# Autodesk Inventor assembly: frame
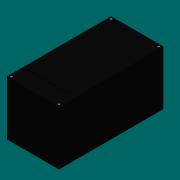
[picture p0: Inventor's stored thumbnail of the model, 180x180]
Saved by Autodesk Inventor 2016 SP1 (Build 200210100, 210)
## iProperties
Created: 2015-10-13
Part Number: frame
Document SubType Name: Assembly
Designer: Sawaiz
Author: Sawaiz
## Documents named in this file (16)
- C:\Users\sawai\OneDrive\projects\modularRICH\frame\frame.iam
- C:\Users\sawai\OneDrive\projects\modularRICH\frame\leftSide.ipt
- C:\Users\sawai\OneDrive\projects\modularRICH\frame\rightSide.ipt
- C:\Users\sawai\OneDrive\projects\modularRICH\frame\back.ipt
- C:\Users\sawai\OneDrive\projects\modularRICH\frame\bottom.ipt
- C:\Users\sawai\OneDrive\projects\modularRICH\frame\front.ipt
- C:\Users\sawai\OneDrive\projects\modularRICH\frame\top.ipt
- C:\Users\sawai\OneDrive\projects\modularRICH\hardware\4-40x0.5in.ipt
- C:\Users\sawai\OneDrive\projects\modularRICH\frame\topORing.ipt
- C:\Users\sawai\OneDrive\projects\modularRICH\dependency\modularRICHBackplane\cad\backplane.iam
- C:\Users\sawai\OneDrive\projects\modularRICH\hardware\no4nut.ipt
- C:\Users\sawai\OneDrive\projects\modularRICH\hardware\no4washer.ipt
- C:\Users\sawai\OneDrive\projects\modularRICH\connector\shv.ipt
- C:\Users\sawai\OneDrive\projects\modularRICH\connector\lvConnector.ipt
- C:\Users\sawai\OneDrive\projects\modularRICH\hardware\4-40x0.325in.ipt
- C:\Users\sawai\OneDrive\projects\modularRICH\modularRICH.xlsx
## Components (46 placed, 14 different names)
1. leftSide:1 — Flush:1, Flush:2, Flush:9, Flush:10
2. rightSide:1 — Flush:1, Flush:2, Flush:3, Flush:4, Flush:5, Mate:2, Flush:8, Mate:3
3. back:1 — Flush:4, Flush:8, Mate:3, Flush:11, Mate:36, Flush:22, Mate:37, Mate:38, Mate:39, Mate:40, Mate:41, Mate:42, Mate:43, Mate:69, Mate:72, Mate:73, Mate:74, Mate:75, Mate:76, Mate:77, Mate:78, Mate:79, Mate:80, Mate:81, Mate:82
4. bottom:1 — Flush:6, Mate:1, Flush:7
5. front:1 — Flush:3, Flush:5, Flush:6, Mate:1, Flush:7, Mate:2, Flush:9, Mate:11
6. top:1 — Flush:10, Flush:11, Mate:4, Mate:5, Mate:6, Mate:7, Flush:12, Flush:13, Flush:14, Flush:15, Mate:8, Mate:9, Mate:10, Mate:11
7. 4-40x0.5in:1 — Mate:4, Flush:15
8. 4-40x0.5in:2 — Mate:7, Flush:12
9. 4-40x0.5in:3 — Mate:6, Flush:13
10. 4-40x0.5in:4 — Mate:5, Flush:14
11. topORing:1 — Mate:8, Mate:9, Mate:10
12. 4-40x0.5in:5 — Mate:36, Flush:22, Flush:28, Flush:29, Mate:46
13. 4-40x0.5in:6 — Mate:37, Flush:29, Mate:66
14. 4-40x0.5in:7 — Mate:38, Flush:23, Mate:67
15. 4-40x0.5in:8 — Mate:42, Flush:27, Flush:28, Mate:62
16. 4-40x0.5in:9 — Mate:39, Flush:25, Flush:26, Mate:64
17. 4-40x0.5in:10 — Mate:40, Flush:26, Flush:27, Mate:63
18. 4-40x0.5in:11 — Mate:41, Flush:24, Flush:25, Mate:65
19. 4-40x0.5in:12 — Mate:43, Flush:23, Flush:24, Mate:68
20. no4nut:1 — Mate:44, Mate:45, Mate:46, Flush:30
21. no4washer:1 — Mate:44, Mate:45
22. no4nut:2 — Mate:64, Flush:35, Flush:36
23. no4washer:2 — Mate:71
24. no4nut:3 — Mate:63, Flush:36, Flush:37
25. no4washer:3
26. no4nut:4 — Mate:65, Flush:34, Flush:35
27. no4washer:4
28. no4nut:5 — Mate:67, Flush:32, Flush:33
29. no4washer:5
30. no4nut:6 — Mate:68, Flush:33, Flush:34
31. no4washer:6
32. no4nut:7 — Mate:66, Flush:31, Flush:32
33. no4washer:7
34. no4nut:8 — Mate:62, Flush:30, Flush:31, Flush:37
35. no4washer:8 — Mate:70
36. backplane:1 [sub-assembly] — Mate:69, Mate:70, Mate:71
37. shv:1 — Mate:72, Mate:73, Flush:38
38. shv:2 — Mate:74, Flush:38, Flush:40
39. shv:3 — Mate:75, Flush:39, Flush:40
40. shv:4 — Mate:76, Flush:39
41. lvConnector:1 — Mate:77, Mate:78, Mate:79, Mate:86, Mate:87, Mate:88, Mate:89
42. lvConnector:2 — Mate:80, Mate:81, Mate:82, Mate:83, Mate:84, Mate:85, Mate:90
43. 4-40x0.325in:1 — Mate:83, Mate:84
44. 4-40x0.325in:2 — Mate:85, Mate:90
45. 4-40x0.325in:3 — Mate:86, Mate:88
46. 4-40x0.325in:4 — Mate:87, Mate:89
## Relationships (99: Mate 65, Flush 34)
- Flush:1: leftSide:1 ↔ rightSide:1
- Flush:2: leftSide:1 ↔ rightSide:1
- Flush:3: rightSide:1 ↔ front:1
- Flush:4: rightSide:1 ↔ back:1
- Flush:5: rightSide:1 ↔ front:1
- Flush:6: bottom:1 ↔ front:1
- Mate:1: bottom:1 ↔ front:1
- Flush:7: bottom:1 ↔ front:1
- Mate:2: rightSide:1 ↔ front:1
- Flush:8: rightSide:1 ↔ back:1
- Mate:3: rightSide:1 ↔ back:1
- Flush:9: leftSide:1 ↔ front:1
- Flush:10: leftSide:1 ↔ top:1
- Flush:11: back:1 ↔ top:1
- Mate:4: top:1 ↔ 4-40x0.5in:1
- Mate:5: top:1 ↔ 4-40x0.5in:4
- Mate:6: top:1 ↔ 4-40x0.5in:3
- Mate:7: top:1 ↔ 4-40x0.5in:2
- Flush:12: top:1 ↔ 4-40x0.5in:2
- Flush:13: top:1 ↔ 4-40x0.5in:3
- Flush:14: top:1 ↔ 4-40x0.5in:4
- Flush:15: top:1 ↔ 4-40x0.5in:1
- Mate:8: top:1 ↔ topORing:1
- Mate:9: top:1 ↔ topORing:1
- Mate:10: top:1 ↔ topORing:1
- Mate:11: front:1 ↔ top:1
- Mate:36: back:1 ↔ 4-40x0.5in:5
- Flush:22: back:1 ↔ 4-40x0.5in:5
- Mate:37: back:1 ↔ 4-40x0.5in:6
- Mate:38: back:1 ↔ 4-40x0.5in:7
- Mate:39: back:1 ↔ 4-40x0.5in:9
- Mate:40: back:1 ↔ 4-40x0.5in:10
- Mate:41: back:1 ↔ 4-40x0.5in:11
- Mate:42: back:1 ↔ 4-40x0.5in:8
- Mate:43: back:1 ↔ 4-40x0.5in:12
- Flush:23: 4-40x0.5in:7 ↔ 4-40x0.5in:12
- Flush:24: 4-40x0.5in:11 ↔ 4-40x0.5in:12
- Flush:25: 4-40x0.5in:9 ↔ 4-40x0.5in:11
- Flush:26: 4-40x0.5in:9 ↔ 4-40x0.5in:10
- Flush:27: 4-40x0.5in:8 ↔ 4-40x0.5in:10
- Flush:28: 4-40x0.5in:5 ↔ 4-40x0.5in:8
- Flush:29: 4-40x0.5in:5 ↔ 4-40x0.5in:6
- Mate:44: no4nut:1 ↔ no4washer:1
- Mate:45: no4nut:1 ↔ no4washer:1
- Mate:46: 4-40x0.5in:5 ↔ no4nut:1
- [Mate]: no4nut:2 ↔ no4washer:2
- [Mate]: no4nut:2 ↔ no4washer:2
- [Mate]: no4nut:3 ↔ no4washer:3
- [Mate]: no4nut:3 ↔ no4washer:3
- [Mate]: no4nut:4 ↔ no4washer:4
- [Mate]: no4nut:4 ↔ no4washer:4
- [Mate]: no4nut:5 ↔ no4washer:5
- [Mate]: no4nut:5 ↔ no4washer:5
- [Mate]: no4nut:6 ↔ no4washer:6
- [Mate]: no4nut:6 ↔ no4washer:6
- [Mate]: no4nut:7 ↔ no4washer:7
- [Mate]: no4nut:7 ↔ no4washer:7
- [Mate]: no4nut:8 ↔ no4washer:8
- [Mate]: no4nut:8 ↔ no4washer:8
- Mate:62: 4-40x0.5in:8 ↔ no4nut:8
- Mate:63: 4-40x0.5in:10 ↔ no4nut:3
- Mate:64: 4-40x0.5in:9 ↔ no4nut:2
- Mate:65: 4-40x0.5in:11 ↔ no4nut:4
- Mate:66: 4-40x0.5in:6 ↔ no4nut:7
- Mate:67: 4-40x0.5in:7 ↔ no4nut:5
- Mate:68: 4-40x0.5in:12 ↔ no4nut:6
- Flush:30: no4nut:1 ↔ no4nut:8
- Flush:31: no4nut:7 ↔ no4nut:8
- Flush:32: no4nut:5 ↔ no4nut:7
- Flush:33: no4nut:5 ↔ no4nut:6
- Flush:34: no4nut:4 ↔ no4nut:6
- Flush:35: no4nut:2 ↔ no4nut:4
- Flush:36: no4nut:2 ↔ no4nut:3
- Flush:37: no4nut:3 ↔ no4nut:8
- Mate:69: back:1 ↔ backplane:1
- Mate:70: no4washer:8 ↔ backplane:1
- Mate:71: no4washer:2 ↔ backplane:1
- Mate:72: back:1 ↔ shv:1
- Mate:73: back:1 ↔ shv:1
- Mate:74: back:1 ↔ shv:2
- Flush:38: shv:1 ↔ shv:2
- Mate:75: back:1 ↔ shv:3
- Mate:76: back:1 ↔ shv:4
- Flush:39: shv:3 ↔ shv:4
- Flush:40: shv:2 ↔ shv:3
- Mate:77: back:1 ↔ lvConnector:1
- Mate:78: back:1 ↔ lvConnector:1
- Mate:79: back:1 ↔ lvConnector:1
- Mate:80: back:1 ↔ lvConnector:2
- Mate:81: back:1 ↔ lvConnector:2
- Mate:82: back:1 ↔ lvConnector:2
- Mate:83: lvConnector:2 ↔ 4-40x0.325in:1
- Mate:84: lvConnector:2 ↔ 4-40x0.325in:1
- Mate:85: lvConnector:2 ↔ 4-40x0.325in:2
- Mate:86: lvConnector:1 ↔ 4-40x0.325in:3
- Mate:87: lvConnector:1 ↔ 4-40x0.325in:4
- Mate:88: lvConnector:1 ↔ 4-40x0.325in:3
- Mate:89: lvConnector:1 ↔ 4-40x0.325in:4
- Mate:90: lvConnector:2 ↔ 4-40x0.325in:2
## Named parameters: acrylicThickness = 6.35 mm, aerogelThickness = 30 mm, height = 127 mm, width = 127 mm, depth = 273.05 mm, mirrorAngle = 5 deg, detectorWidth = 52 mm, detectorHeight = 52 mm, mirrorThickness = 3.175 mm, fresnelThickness = 0.1 mm, grooveDensity = 100, focalLength = 76.2 mm, ior = 1.49, centerThickness = 1.524 mm, fresnelAngle = 90 deg, fresnelEffectiveDiameter = 152.4 mm, mirrorSuppourtWidth = 38.1 mm, backGrooveBit = 4.8006 mm, sensorHolderWidth = 88.9 mm, sensorHolderSensorWidth = 53.975 mm, sensorHolderSesnorHeight = 53.975 mm, sensorHolderHeight = 88.9 mm, sensorHolderSensorHeight = 53.975 mm, sensorHolderORingGroove = 3.175 mm, sensorHolderORing = 3.175 mm, sensorHolderFlushORingID = 304.8 mm, sensorHolderFlushORing = 3.175 mm, frontBackORingID = 419.1 mm, oRingWidth = 1.5875 mm, sensorHolderORingID = 203.2 mm, topBottomHorizontalMirrorGroove = 12.7 mm, backMirrorGroove = 6.35 mm, mirrorGroove = 19.05 mm, compressionPercent = 40, fresnelChamfer = 6.35 mm, mirrorGrooveFillet = 6.35 mm, mirrorGrooveDrill = 6.35 mm, mirrorGrooveMill = 3.175 mm, fresnelMirrorChamfer = 6.35 mm, detectorOpeningHeight = 76.2 mm, detectorOpeningWidth = 76.2 mm, sensorHolderDepth = 19.05 mm, frameAcrylicThickness = 9.525 mm, internalAcrylicThicnkess = 6.35 mm, aerogelWidth = 110 mm, aerogelHeight = 110 mm, internalAcrylicThickness = 6.35 mm, aerogelClearence = 3.175 mm, backplanePCBHeight = 76.2 mm, backplaneHoleOffsett = 6.35 mm, backplanePCBWidth = 76.2 mm, backplanePostionOffsett = 12.7 mm, d277_d273 = 0 mm, d278_d274 = 0 mm, d279_d273 = 0 mm, d280_d274 = 0 mm, d281_d273 = 0 mm, d282_d274 = 0 mm, d283_d273 = 0 mm, d284_d274 = 0 mm, d285_d273 = 0 mm, d286_d274 = 0 mm, d287_d273 = 0 mm, d288_d274 = 0 mm, d289_d273 = 0 mm, d290_d274 = 0 mm, moduleSlotClearence = 0.79375 mm, testMountWidth = 300 mm, testMountHeight = 300 mm, testMountLength = 500 mm
